# Autodesk Inventor assembly: 3D_PCB4_2024-01-15
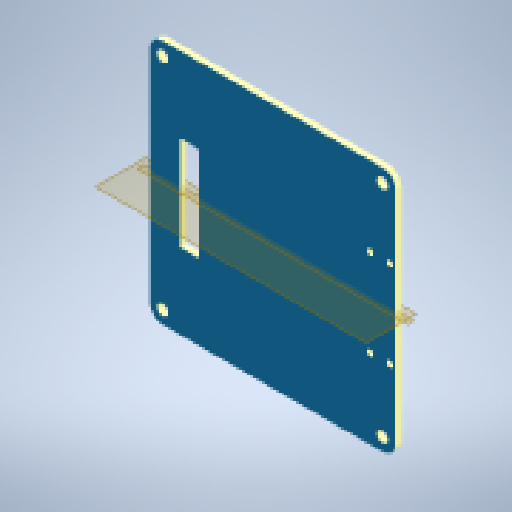
[picture p0: Inventor's stored thumbnail of the model, 512x512]
Saved by Autodesk Inventor 2024.2 (Build 282272000, 272)
## iProperties
Created: 2025-09-19
Part Number: 3D_PCB4_2024-01-15
Document SubType Name: Assembly
Designer: AdminForWorker
Title: 3D_PCB4_2024-01-15 v3
Author: AdminForWorker
## Documents named in this file (2)
- D:\dog\fox\construction\fox\boards\3D_PCB4_2024-01-15 v3.iam
- D:\dog\fox\construction\fox\boards\Board.ipt
## Components (1 placed, 1 different names)
1. Board:1 — Угол:1
## Relationships (1: Angle 1)
- Угол:1 [Angle] (0 deg): Board:1
